# Autodesk Inventor assembly: Assembly1
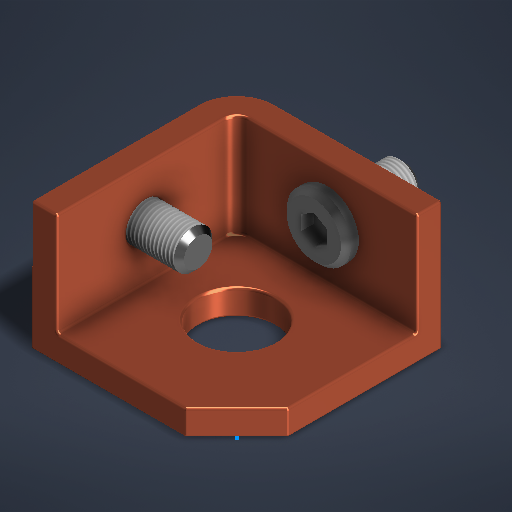
[picture p0: Inventor's stored thumbnail of the model, 512x512]
Saved by Autodesk Inventor 2026.2 (Build 302298000, 298)
## iProperties
Created: 2025-12-08
Part Number: Assembly1
Document SubType Name: Assembly
Designer: Thoma
Author: Thoma
## Documents named in this file (3)
- C:\Users\Thoma\OneDrive\Desktop\Inventor\Learning\Assembly1.iam
- C:\Users\Thoma\OneDrive\Desktop\Inventor\Learning\Part3.ipt
- C:\Users\Thoma\OneDrive\Desktop\Inventor\Learning\Part4.ipt
## Components (3 placed, 2 different names)
1. Part3:1 — Mate:1, Mate:2, Angle:1, Mate:3, Mate:4, Angle:2
2. Part4:1 — Mate:1, Mate:2, Angle:1
3. Part4:2 — Mate:3, Mate:4, Angle:2
## Relationships (6: Mate 4, Angle 2)
- Mate:1: Part3:1 ↔ Part4:1
- Mate:2: Part3:1 ↔ Part4:1
- Angle:1 (0 deg): Part3:1 ↔ Part4:1
- Mate:3: Part3:1 ↔ Part4:2
- Mate:4: Part3:1 ↔ Part4:2
- Angle:2 (0 deg): Part3:1 ↔ Part4:2
